# Autodesk Inventor assembly: ギアボックス片側
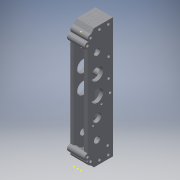
[picture p0: Inventor's stored thumbnail of the model, 180x180]
Saved by Autodesk Inventor 2018 (Build 220112000, 112)
## iProperties
Created: 2018-08-16
Part Number: ギアボックス片側
Material: 一般
Document SubType Name: Assembly
Designer: shun2
Author: shun2
## Documents named in this file (4)
- C:\Users\shun2\OneDrive\おそらく最新版(2018.7.31)\ギアボックス\ギアボックス片側.iam
- C:\Users\shun2\OneDrive\おそらく最新版(2018.7.31)\ギアボックス\1枚目\1枚目.ipt
- C:\Users\shun2\OneDrive\おそらく最新版(2018.7.31)\ギアボックス\2~4枚目\2-4枚目.ipt
- C:\Users\shun2\OneDrive\おそらく最新版(2018.7.31)\ギアボックス\5枚目\5枚目.ipt
## Components (5 placed, 3 different names)
1. 1枚目:1 — メイト:4
2. 5枚目:1 — メイト:1
3. 2-4枚目:1 — メイト:1, メイト:2
4. 2-4枚目:2 — メイト:2, メイト:3
5. 2-4枚目:3 — メイト:3, メイト:4
## Relationships (4: Mate 4)
- メイト:1 [Mate]: 5枚目:1 ↔ 2-4枚目:1
- メイト:2 [Mate]: 2-4枚目:1 ↔ 2-4枚目:2
- メイト:3 [Mate]: 2-4枚目:2 ↔ 2-4枚目:3
- メイト:4 [Mate]: 1枚目:1 ↔ 2-4枚目:3
